# Autodesk Inventor assembly: Ensamblaje4
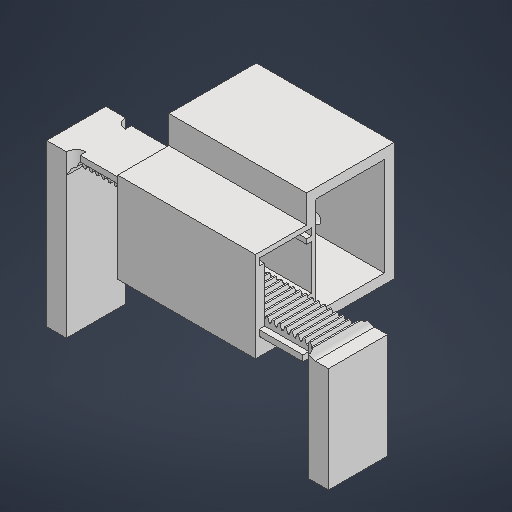
[picture p0: Inventor's stored thumbnail of the model, 512x512]
Saved by Autodesk Inventor 2025.3 (Build 293356000, 356)
## iProperties
Created: 2025-10-14
Part Number: Ensamblaje4
Document SubType Name: Assembly
Designer: Jonathan Galarza
Author: Jonathan Galarza
## Documents named in this file (6)
- D:\ESPE MECATRONICA\TESIS\GARRA\Ensamblaje4.iam
- D:\ESPE MECATRONICA\TESIS\GARRA\cremallera 4.ipt
- D:\ESPE MECATRONICA\TESIS\GARRA\piñon 4.ipt
- D:\ESPE MECATRONICA\TESIS\GARRA\cremallera 4 - copia.ipt
- D:\ESPE MECATRONICA\TESIS\GARRA\baseGuias.ipt
- D:\ESPE MECATRONICA\TESIS\GARRA\stepper-motor-28byj-48-5v-dc-1.snapshot.1\Stepper 28BYJ48\Stepper 28BYJ48\Stepper 28BYJ48.ipt
## Components (5 placed, 5 different names)
1. cremallera 4:1 — Nivelación:2, Nivelación:4, Rotación/Traslación:2, Coincidencia:4
2. piñon 4:1 — Coincidencia:1, Nivelación:1, Nivelación:2, Nivelación:5, Rotación/Traslación:1, Rotación/Traslación:2, Coincidencia:3
3. cremallera 4 - copia:1 — Nivelación:5, Coincidencia:2, Rotación/Traslación:1
4. baseGuias:1 — Coincidencia:3, Coincidencia:4, Coincidencia:5, Coincidencia:6, Coincidencia:7, Coincidencia:8
5. Stepper 28BYJ48:1 — Coincidencia:6, Coincidencia:7, Coincidencia:8
## Relationships (16: Mate 8, Flush 6, RelateRotateTranslate 2)
- Coincidencia:1 [Mate]: piñon 4:1
- Nivelación:1 [Flush]: piñon 4:1
- Nivelación:2 [Flush]: cremallera 4:1 ↔ piñon 4:1
- Nivelación:3 [Flush] (-13 mm)
- Nivelación:4 [Flush]: cremallera 4:1
- Nivelación:5 [Flush]: piñon 4:1 ↔ cremallera 4 - copia:1
- Nivelación:6 [Flush] (13 mm)
- Coincidencia:2 [Mate]: cremallera 4 - copia:1
- Rotación/Traslación:1 [RelateRotateTranslate] (62.8 mm): piñon 4:1 ↔ cremallera 4 - copia:1
- Rotación/Traslación:2 [RelateRotateTranslate] (62.8 mm): cremallera 4:1 ↔ piñon 4:1
- Coincidencia:3 [Mate]: piñon 4:1 ↔ baseGuias:1
- Coincidencia:4 [Mate]: cremallera 4:1 ↔ baseGuias:1
- Coincidencia:5 [Mate]: baseGuias:1
- Coincidencia:6 [Mate]: baseGuias:1 ↔ Stepper 28BYJ48:1
- Coincidencia:7 [Mate]: baseGuias:1 ↔ Stepper 28BYJ48:1
- Coincidencia:8 [Mate]: baseGuias:1 ↔ Stepper 28BYJ48:1
